# Autodesk Inventor assembly: ie-track-kit-pwr-1
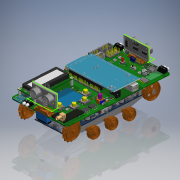
[picture p0: Inventor's stored thumbnail of the model, 180x180]
Saved by Autodesk Inventor 2019.1 (Build 231200000, 200)
## iProperties
Company: Open CASCADE
Created: 2019-03-19
Part Number: ie-track-kit-pwr-1
Description: Open CASCADE Model
Document SubType Name: Assembly
Designer: poryz
Authority: Unknown
Sending System: Open CASCADE 6.8
Preprocessor: Open CASCADE STEP processor 6.8
Title: Open CASCADE Shape Model
Author: Author
## Documents named in this file (135)
- E:\Dropbox\_UCZELNIA\___ARTYKULY\badania\KKE2019\inventor\ie-track-kit-pwr-1.iam
- E:\Dropbox\_UCZELNIA\___ARTYKULY\badania\KKE2019\inventor\Board.ipt
- E:\Dropbox\_UCZELNIA\___ARTYKULY\badania\KKE2019\inventor\R11.iam
- E:\Dropbox\_UCZELNIA\___ARTYKULY\badania\KKE2019\inventor\Q4.iam
- E:\Dropbox\_UCZELNIA\___ARTYKULY\badania\KKE2019\inventor\Q3.iam
- E:\Dropbox\_UCZELNIA\___ARTYKULY\badania\KKE2019\inventor\2.iam
- E:\Dropbox\_UCZELNIA\___ARTYKULY\badania\KKE2019\inventor\R21.iam
- E:\Dropbox\_UCZELNIA\___ARTYKULY\badania\KKE2019\inventor\D4.iam
- E:\Dropbox\_UCZELNIA\___ARTYKULY\badania\KKE2019\inventor\C3.iam
- E:\Dropbox\_UCZELNIA\___ARTYKULY\badania\KKE2019\inventor\BT1.iam
- E:\Dropbox\_UCZELNIA\___ARTYKULY\badania\KKE2019\inventor\R9.iam
- E:\Dropbox\_UCZELNIA\___ARTYKULY\badania\KKE2019\inventor\R8.iam
- E:\Dropbox\_UCZELNIA\___ARTYKULY\badania\KKE2019\inventor\R10.iam
- E:\Dropbox\_UCZELNIA\___ARTYKULY\badania\KKE2019\inventor\R7.iam
- E:\Dropbox\_UCZELNIA\___ARTYKULY\badania\KKE2019\inventor\Q2.iam
- E:\Dropbox\_UCZELNIA\___ARTYKULY\badania\KKE2019\inventor\D1.iam
- E:\Dropbox\_UCZELNIA\___ARTYKULY\badania\KKE2019\inventor\C5.iam
- E:\Dropbox\_UCZELNIA\___ARTYKULY\badania\KKE2019\inventor\C4.iam
- E:\Dropbox\_UCZELNIA\___ARTYKULY\badania\KKE2019\inventor\BT3.iam
- E:\Dropbox\_UCZELNIA\___ARTYKULY\badania\KKE2019\inventor\GND1.iam
- E:\Dropbox\_UCZELNIA\___ARTYKULY\badania\KKE2019\inventor\3.iam
- E:\Dropbox\_UCZELNIA\___ARTYKULY\badania\KKE2019\inventor\1.iam
- E:\Dropbox\_UCZELNIA\___ARTYKULY\badania\KKE2019\inventor\R16.iam
- E:\Dropbox\_UCZELNIA\___ARTYKULY\badania\KKE2019\inventor\P1.iam
- E:\Dropbox\_UCZELNIA\___ARTYKULY\badania\KKE2019\inventor\D9.iam
- E:\Dropbox\_UCZELNIA\___ARTYKULY\badania\KKE2019\inventor\D8.iam
- E:\Dropbox\_UCZELNIA\___ARTYKULY\badania\KKE2019\inventor\R31.iam
- E:\Dropbox\_UCZELNIA\___ARTYKULY\badania\KKE2019\inventor\R20.iam
- E:\Dropbox\_UCZELNIA\___ARTYKULY\badania\KKE2019\inventor\MH5.iam
- E:\Dropbox\_UCZELNIA\___ARTYKULY\badania\KKE2019\inventor\MH9.iam
- E:\Dropbox\_UCZELNIA\___ARTYKULY\badania\KKE2019\inventor\MH11.iam
- E:\Dropbox\_UCZELNIA\___ARTYKULY\badania\KKE2019\inventor\BT2.iam
- E:\Dropbox\_UCZELNIA\___ARTYKULY\badania\KKE2019\inventor\D6.iam
- E:\Dropbox\_UCZELNIA\___ARTYKULY\badania\KKE2019\inventor\Q7.iam
- E:\Dropbox\_UCZELNIA\___ARTYKULY\badania\KKE2019\inventor\Q18.iam
- E:\Dropbox\_UCZELNIA\___ARTYKULY\badania\KKE2019\inventor\Q16.iam
- E:\Dropbox\_UCZELNIA\___ARTYKULY\badania\KKE2019\inventor\Q14.iam
- E:\Dropbox\_UCZELNIA\___ARTYKULY\badania\KKE2019\inventor\R43.iam
- E:\Dropbox\_UCZELNIA\___ARTYKULY\badania\KKE2019\inventor\R42.iam
- E:\Dropbox\_UCZELNIA\___ARTYKULY\badania\KKE2019\inventor\R41.iam
- E:\Dropbox\_UCZELNIA\___ARTYKULY\badania\KKE2019\inventor\R40.iam
- E:\Dropbox\_UCZELNIA\___ARTYKULY\badania\KKE2019\inventor\Q17.iam
- E:\Dropbox\_UCZELNIA\___ARTYKULY\badania\KKE2019\inventor\Q15.iam
- E:\Dropbox\_UCZELNIA\___ARTYKULY\badania\KKE2019\inventor\SW1.iam
- E:\Dropbox\_UCZELNIA\___ARTYKULY\badania\KKE2019\inventor\D18.iam
- E:\Dropbox\_UCZELNIA\___ARTYKULY\badania\KKE2019\inventor\D19.iam
- E:\Dropbox\_UCZELNIA\___ARTYKULY\badania\KKE2019\inventor\D17.iam
- E:\Dropbox\_UCZELNIA\___ARTYKULY\badania\KKE2019\inventor\D16.iam
- E:\Dropbox\_UCZELNIA\___ARTYKULY\badania\KKE2019\inventor\D15.iam
- E:\Dropbox\_UCZELNIA\___ARTYKULY\badania\KKE2019\inventor\D14.iam
- E:\Dropbox\_UCZELNIA\___ARTYKULY\badania\KKE2019\inventor\R32.iam
- E:\Dropbox\_UCZELNIA\___ARTYKULY\badania\KKE2019\inventor\R33.iam
- E:\Dropbox\_UCZELNIA\___ARTYKULY\badania\KKE2019\inventor\R30.iam
- E:\Dropbox\_UCZELNIA\___ARTYKULY\badania\KKE2019\inventor\Q9.iam
- E:\Dropbox\_UCZELNIA\___ARTYKULY\badania\KKE2019\inventor\Q10.iam
- E:\Dropbox\_UCZELNIA\___ARTYKULY\badania\KKE2019\inventor\D11.iam
- E:\Dropbox\_UCZELNIA\___ARTYKULY\badania\KKE2019\inventor\D10.iam
- E:\Dropbox\_UCZELNIA\___ARTYKULY\badania\KKE2019\inventor\C17.iam
- E:\Dropbox\_UCZELNIA\___ARTYKULY\badania\KKE2019\inventor\D5.iam
- E:\Dropbox\_UCZELNIA\___ARTYKULY\badania\KKE2019\inventor\MH10.iam
- E:\Dropbox\_UCZELNIA\___ARTYKULY\badania\KKE2019\inventor\MH7.iam
- E:\Dropbox\_UCZELNIA\___ARTYKULY\badania\KKE2019\inventor\MH6.iam
- E:\Dropbox\_UCZELNIA\___ARTYKULY\badania\KKE2019\inventor\C20.iam
- E:\Dropbox\_UCZELNIA\___ARTYKULY\badania\KKE2019\inventor\U1.iam
- E:\Dropbox\_UCZELNIA\___ARTYKULY\badania\KKE2019\inventor\R5.iam
- E:\Dropbox\_UCZELNIA\___ARTYKULY\badania\KKE2019\inventor\R4.iam
- E:\Dropbox\_UCZELNIA\___ARTYKULY\badania\KKE2019\inventor\R3.iam
- E:\Dropbox\_UCZELNIA\___ARTYKULY\badania\KKE2019\inventor\R2.iam
- E:\Dropbox\_UCZELNIA\___ARTYKULY\badania\KKE2019\inventor\R1.iam
- E:\Dropbox\_UCZELNIA\___ARTYKULY\badania\KKE2019\inventor\Q1.iam
- E:\Dropbox\_UCZELNIA\___ARTYKULY\badania\KKE2019\inventor\C2.iam
- E:\Dropbox\_UCZELNIA\___ARTYKULY\badania\KKE2019\inventor\C1.iam
- E:\Dropbox\_UCZELNIA\___ARTYKULY\badania\KKE2019\inventor\C6.iam
- E:\Dropbox\_UCZELNIA\___ARTYKULY\badania\KKE2019\inventor\U2.iam
- E:\Dropbox\_UCZELNIA\___ARTYKULY\badania\KKE2019\inventor\R15.iam
- E:\Dropbox\_UCZELNIA\___ARTYKULY\badania\KKE2019\inventor\R19.iam
- E:\Dropbox\_UCZELNIA\___ARTYKULY\badania\KKE2019\inventor\R12.iam
- E:\Dropbox\_UCZELNIA\___ARTYKULY\badania\KKE2019\inventor\SW2.iam
- E:\Dropbox\_UCZELNIA\___ARTYKULY\badania\KKE2019\inventor\L1.iam
- E:\Dropbox\_UCZELNIA\___ARTYKULY\badania\KKE2019\inventor\D3.iam
- E:\Dropbox\_UCZELNIA\___ARTYKULY\badania\KKE2019\inventor\C7.iam
- E:\Dropbox\_UCZELNIA\___ARTYKULY\badania\KKE2019\inventor\C8.iam
- E:\Dropbox\_UCZELNIA\___ARTYKULY\badania\KKE2019\inventor\C10.iam
- E:\Dropbox\_UCZELNIA\___ARTYKULY\badania\KKE2019\inventor\C9.iam
- E:\Dropbox\_UCZELNIA\___ARTYKULY\badania\KKE2019\inventor\C11.iam
- E:\Dropbox\_UCZELNIA\___ARTYKULY\badania\KKE2019\inventor\Q5.iam
- E:\Dropbox\_UCZELNIA\___ARTYKULY\badania\KKE2019\inventor\Q8.iam
- E:\Dropbox\_UCZELNIA\___ARTYKULY\badania\KKE2019\inventor\R13.iam
- E:\Dropbox\_UCZELNIA\___ARTYKULY\badania\KKE2019\inventor\R18.iam
- E:\Dropbox\_UCZELNIA\___ARTYKULY\badania\KKE2019\inventor\R17.iam
- E:\Dropbox\_UCZELNIA\___ARTYKULY\badania\KKE2019\inventor\C12.iam
- E:\Dropbox\_UCZELNIA\___ARTYKULY\badania\KKE2019\inventor\C13.iam
- E:\Dropbox\_UCZELNIA\___ARTYKULY\badania\KKE2019\inventor\C14.iam
- E:\Dropbox\_UCZELNIA\___ARTYKULY\badania\KKE2019\inventor\C15.iam
- E:\Dropbox\_UCZELNIA\___ARTYKULY\badania\KKE2019\inventor\C16.iam
- E:\Dropbox\_UCZELNIA\___ARTYKULY\badania\KKE2019\inventor\D7.iam
- E:\Dropbox\_UCZELNIA\___ARTYKULY\badania\KKE2019\inventor\L2.iam
- E:\Dropbox\_UCZELNIA\___ARTYKULY\badania\KKE2019\inventor\R23.iam
- E:\Dropbox\_UCZELNIA\___ARTYKULY\badania\KKE2019\inventor\R24.iam
- E:\Dropbox\_UCZELNIA\___ARTYKULY\badania\KKE2019\inventor\R26.iam
- E:\Dropbox\_UCZELNIA\___ARTYKULY\badania\KKE2019\inventor\R27.iam
- E:\Dropbox\_UCZELNIA\___ARTYKULY\badania\KKE2019\inventor\R28.iam
- E:\Dropbox\_UCZELNIA\___ARTYKULY\badania\KKE2019\inventor\R29.iam
- E:\Dropbox\_UCZELNIA\___ARTYKULY\badania\KKE2019\inventor\U3.iam
- E:\Dropbox\_UCZELNIA\___ARTYKULY\badania\KKE2019\inventor\R22.iam
- E:\Dropbox\_UCZELNIA\___ARTYKULY\badania\KKE2019\inventor\D2.iam
- E:\Dropbox\_UCZELNIA\___ARTYKULY\badania\KKE2019\inventor\R14.iam
- E:\Dropbox\_UCZELNIA\___ARTYKULY\badania\KKE2019\inventor\R25.iam
- E:\Dropbox\_UCZELNIA\___ARTYKULY\badania\KKE2019\inventor\U4.iam
- E:\Dropbox\_UCZELNIA\___ARTYKULY\badania\KKE2019\inventor\U5.iam
- E:\Dropbox\_UCZELNIA\___ARTYKULY\badania\KKE2019\inventor\C22.iam
- E:\Dropbox\_UCZELNIA\___ARTYKULY\badania\KKE2019\inventor\C21.iam
- E:\Dropbox\_UCZELNIA\___ARTYKULY\badania\KKE2019\inventor\C19.iam
- E:\Dropbox\_UCZELNIA\___ARTYKULY\badania\KKE2019\inventor\C18.iam
- E:\Dropbox\_UCZELNIA\___ARTYKULY\badania\KKE2019\inventor\R6.iam
- E:\Dropbox\_UCZELNIA\___ARTYKULY\badania\KKE2019\inventor\Q6.iam
- E:\Dropbox\_UCZELNIA\___ARTYKULY\badania\KKE2019\inventor\CN2.iam
- E:\Dropbox\_UCZELNIA\___ARTYKULY\badania\KKE2019\inventor\Q13.iam
- E:\Dropbox\_UCZELNIA\___ARTYKULY\badania\KKE2019\inventor\R38.iam
- E:\Dropbox\_UCZELNIA\___ARTYKULY\badania\KKE2019\inventor\R39.iam
- E:\Dropbox\_UCZELNIA\___ARTYKULY\badania\KKE2019\inventor\D12.iam
- E:\Dropbox\_UCZELNIA\___ARTYKULY\badania\KKE2019\inventor\D13.iam
- E:\Dropbox\_UCZELNIA\___ARTYKULY\badania\KKE2019\inventor\D20.iam
- E:\Dropbox\_UCZELNIA\___ARTYKULY\badania\KKE2019\inventor\D21.iam
- E:\Dropbox\_UCZELNIA\___ARTYKULY\badania\KKE2019\inventor\D23.iam
- E:\Dropbox\_UCZELNIA\___ARTYKULY\badania\KKE2019\inventor\D22.iam
- E:\Dropbox\_UCZELNIA\___ARTYKULY\badania\KKE2019\inventor\Q12.iam
- E:\Dropbox\_UCZELNIA\___ARTYKULY\badania\KKE2019\inventor\Q11.iam
- E:\Dropbox\_UCZELNIA\___ARTYKULY\badania\KKE2019\inventor\R37.iam
- E:\Dropbox\_UCZELNIA\___ARTYKULY\badania\KKE2019\inventor\R35.iam
- E:\Dropbox\_UCZELNIA\___ARTYKULY\badania\KKE2019\inventor\R34.iam
- E:\Dropbox\_UCZELNIA\___ARTYKULY\badania\KKE2019\inventor\R36.iam
- E:\Dropbox\_UCZELNIA\___ARTYKULY\badania\KKE2019\inventor\Free-Models.iam
- E:\Dropbox\_UCZELNIA\___ARTYKULY\badania\KKE2019\inventor\line_sensor\line_sensor.iam
- E:\Dropbox\_UCZELNIA\___ARTYKULY\badania\KKE2019\inventor\upper_deck\ie-track-kit-arduino-1-V11.iam
## Components (134 placed, 134 different names)
1. Board_2419
2. R11_2421 [sub-assembly]
3. Q4_2423 [sub-assembly]
4. Q3_2425 [sub-assembly]
5. 2_2429 [sub-assembly]
6. R21_2431 [sub-assembly]
7. D4_2433 [sub-assembly]
8. C3_2435 [sub-assembly]
9. BT1_2439 [sub-assembly]
10. R9_2441 [sub-assembly]
11. R8_2443 [sub-assembly]
12. R10_2445 [sub-assembly]
13. R7_2447 [sub-assembly]
14. Q2_2449 [sub-assembly]
15. D1_2451 [sub-assembly]
16. C5_2453 [sub-assembly]
17. C4_2455 [sub-assembly]
18. BT3_2459 [sub-assembly]
19. GND1_2463 [sub-assembly]
20. 3_2465 [sub-assembly]
21. 1_2467 [sub-assembly]
22. R16_2469 [sub-assembly]
23. P1_2472 [sub-assembly]
24. D9_2485 [sub-assembly]
25. D8_2487 [sub-assembly]
26. R31_2489 [sub-assembly]
27. R20_2491 [sub-assembly]
28. MH5_2493 [sub-assembly]
29. MH9_2495 [sub-assembly]
30. MH11_2497 [sub-assembly]
31. BT2_2501 [sub-assembly]
32. D6_2503 [sub-assembly]
33. Q7_2505 [sub-assembly]
34. Q18_2507 [sub-assembly]
35. Q16_2509 [sub-assembly]
36. Q14_2511 [sub-assembly]
37. R43_2513 [sub-assembly]
38. R42_2515 [sub-assembly]
39. R41_2517 [sub-assembly]
40. R40_2519 [sub-assembly]
41. Q17_2521 [sub-assembly]
42. Q15_2523 [sub-assembly]
43. SW1_2525 [sub-assembly]
44. D18_2528 [sub-assembly]
45. D19_2530 [sub-assembly]
46. D17_2532 [sub-assembly]
47. D16_2534 [sub-assembly]
48. D15_2536 [sub-assembly]
49. D14_2538 [sub-assembly]
50. R32_2540 [sub-assembly]
51. R33_2542 [sub-assembly]
52. R30_2544 [sub-assembly]
53. Q9_2546 [sub-assembly]
54. Q10_2548 [sub-assembly]
55. D11_2550 [sub-assembly]
56. D10_2552 [sub-assembly]
57. C17_2558 [sub-assembly]
58. D5_2560 [sub-assembly]
59. MH10_2562 [sub-assembly]
60. MH7_2564 [sub-assembly]
61. MH6_2566 [sub-assembly]
62. C20_2568 [sub-assembly]
63. U1_2570 [sub-assembly]
64. R5_2572 [sub-assembly]
65. R4_2574 [sub-assembly]
66. R3_2576 [sub-assembly]
67. R2_2578 [sub-assembly]
68. R1_2580 [sub-assembly]
69. Q1_2582 [sub-assembly]
70. C2_2584 [sub-assembly]
71. C1_2586 [sub-assembly]
72. C6_2588 [sub-assembly]
73. U2_2590 [sub-assembly]
74. R15_2592 [sub-assembly]
75. R19_2594 [sub-assembly]
76. R12_2596 [sub-assembly]
77. SW2_2603 [sub-assembly]
78. L1_2608 [sub-assembly]
79. D3_2610 [sub-assembly]
80. C7_2612 [sub-assembly]
81. C8_2614 [sub-assembly]
82. C10_2616 [sub-assembly]
83. C9_2618 [sub-assembly]
84. C11_2620 [sub-assembly]
85. Q5_2622 [sub-assembly]
86. Q8_2624 [sub-assembly]
87. R13_2626 [sub-assembly]
88. R18_2628 [sub-assembly]
89. R17_2630 [sub-assembly]
90. C12_2632 [sub-assembly]
91. C13_2634 [sub-assembly]
92. C14_2636 [sub-assembly]
93. C15_2638 [sub-assembly]
94. C16_2640 [sub-assembly]
95. D7_2642 [sub-assembly]
96. L2_2644 [sub-assembly]
97. R23_2646 [sub-assembly]
98. R24_2648 [sub-assembly]
99. R26_2650 [sub-assembly]
100. R27_2652 [sub-assembly]
101. R28_2654 [sub-assembly]
102. R29_2656 [sub-assembly]
103. U3_2658 [sub-assembly]
104. R22_2660 [sub-assembly]
105. D2_2662 [sub-assembly]
106. R14_2664 [sub-assembly]
107. R25_2666 [sub-assembly]
108. U4_2669 [sub-assembly]
109. U5_2671 [sub-assembly]
110. C22_2673 [sub-assembly]
111. C21_2675 [sub-assembly]
112. C19_2677 [sub-assembly]
113. C18_2679 [sub-assembly]
114. R6_2681 [sub-assembly]
115. Q6_2683 [sub-assembly]
116. CN2_2742 [sub-assembly]
117. Q13_2744 [sub-assembly]
118. R38_2746 [sub-assembly]
119. R39_2748 [sub-assembly]
120. D12_2750 [sub-assembly]
121. D13_2752 [sub-assembly]
122. D20_2754 [sub-assembly]
123. D21_2756 [sub-assembly]
124. D23_2758 [sub-assembly]
125. D22_2760 [sub-assembly]
126. Q12_2762 [sub-assembly]
127. Q11_2764 [sub-assembly]
128. R37_2766 [sub-assembly]
129. R35_2768 [sub-assembly]
130. R34_2770 [sub-assembly]
131. R36_2772 [sub-assembly]
132. Free-Models_2838 [sub-assembly] — Mate:1, Mate:2, Mate:3, Mate:4, Mate:5
133. line_sensor:1 [sub-assembly] — Mate:1, Mate:2, Mate:3
134. ie-track-kit-arduino-1-V11:1 [sub-assembly] — Mate:4, Mate:5
## Relationships (5: Mate 5)
- Mate:1: Free-Models_2838 ↔ line_sensor:1
- Mate:2 (0.5 mm): Free-Models_2838 ↔ line_sensor:1
- Mate:3 (0.5 mm): Free-Models_2838 ↔ line_sensor:1
- Mate:4: Free-Models_2838 ↔ ie-track-kit-arduino-1-V11:1
- Mate:5 (1 mm): Free-Models_2838 ↔ ie-track-kit-arduino-1-V11:1
